# Autodesk Inventor assembly: TableGears
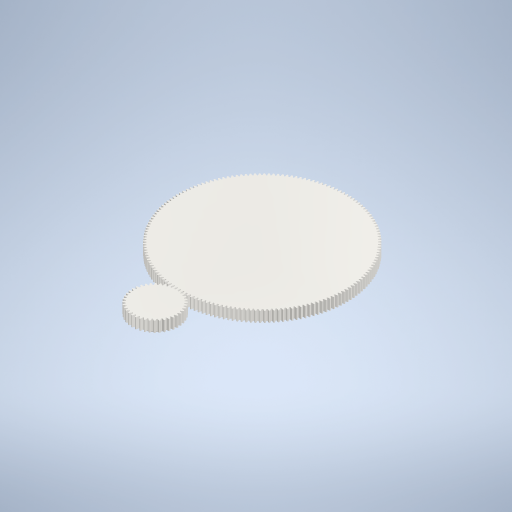
[picture p0: Inventor's stored thumbnail of the model, 512x512]
Saved by Autodesk Inventor 2023 (Build 270158000, 158)
## iProperties
Created: 2023-04-03
Part Number: TableGears
Document SubType Name: Assembly
Designer: czapa
Author: czapa
## Documents named in this file (4)
- C:\Users\czapa\OneDrive\Documents\GitHub\S.P.I.C.E\3D Models\Version1\TableGears.iam
- C:\Users\czapa\OneDrive\Documents\GitHub\S.P.I.C.E\3D Models\Version1\BearingTableGear.ipt
- C:\Users\czapa\OneDrive\Documents\GitHub\S.P.I.C.E\3D Models\Version1\motor_gearMK2.ipt
- C:\Users\czapa\OneDrive\Documents\GitHub\S.P.I.C.E\3D Models\Version1\TableGears\Design Accelerator\Spur Gears1.iam
## Components (3 placed, 3 different names)
1. BearingTableGear:1 — Tangent:1, Flush:1, Mate:3
2. motor_gearMK2:1 — Tangent:1, Flush:1, Mate:1, Mate:2
3. Spur Gears:1 [sub-assembly] — Mate:1, Mate:2, Mate:3
## Relationships (5: Mate 3, Tangent 1, Flush 1)
- Tangent:1 (50 mm): BearingTableGear:1 ↔ motor_gearMK2:1
- Flush:1: BearingTableGear:1 ↔ motor_gearMK2:1
- Mate:1: motor_gearMK2:1 ↔ Spur Gears:1
- Mate:2: motor_gearMK2:1 ↔ Spur Gears:1
- Mate:3: BearingTableGear:1 ↔ Spur Gears:1
